# Autodesk Inventor assembly: Wheel_and_Tire
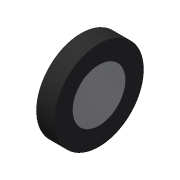
[picture p0: Inventor's stored thumbnail of the model, 180x180]
Saved by Autodesk Inventor 2018 (Build 220112000, 112)
## iProperties
Created: 2017-08-21
Part Number: Wheel_and_Tire
Document SubType Name: Assembly
Designer: thoma
Author: thoma
## Documents named in this file (3)
- C:\Users\thoma\Desktop\Tiny_House\Trailer\Wheel_and_Tire.iam
- C:\Users\thoma\Desktop\Tiny_House\Trailer\Wheel.ipt
- C:\Users\thoma\Desktop\Tiny_House\Trailer\Tire.ipt
## Components (2 placed, 2 different names)
1. Wheel:1 — Insert:1
2. Tire:1 — Insert:1
## Relationships (1: Insert 1)
- Insert:1: Wheel:1 ↔ Tire:1
